# Autodesk Inventor assembly: x_carryage
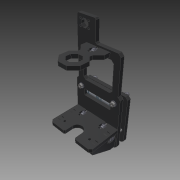
[picture p0: Inventor's stored thumbnail of the model, 180x180]
Saved by Autodesk Inventor 2014 (Build 180170000, 170)
## iProperties
Created: 2014-01-10
Part Number: x_carryage
Document SubType Name: Assembly
Designer: buben
Author: buben
## Documents named in this file (12)
- C:\Users\buben\Documents\GitHub\bacon\inventor files\assemblies\x_carryage.iam
- C:\Users\buben\Documents\GitHub\bacon\inventor files\printer parts\x_carriage_front.ipt
- C:\Users\buben\Documents\GitHub\bacon\inventor files\3rd party components\linear_bearing_8\Imported Components\LU8MM\LU8MM.iam
- C:\Users\buben\Documents\GitHub\bacon\inventor files\printer parts\x_carriage_back.ipt
- C:\Users\buben\Documents\GitHub\bacon\inventor files\printer parts\x_carriage_extruder_mount.ipt
- C:\Users\buben\Documents\GitHub\bacon\inventor files\printer parts\x_carryage_brace.ipt
- C:\Users\buben\Documents\GitHub\bacon\inventor files\printer parts\filament_guide.ipt
- C:\Users\buben\Documents\GitHub\bacon\inventor files\utils\washer_m4.ipt
- C:\Users\buben\Documents\Inventor\Content Center Files\R2014\en-US\ISO 4762(2)\ISO 4762 - M4 x 20ISO.ipt
- C:\Users\buben\Documents\Inventor\Content Center Files\R2014\en-US\ISO 4762(2)\ISO 4762 - M4 x 35ISO.ipt
- C:\Users\buben\Documents\Inventor\Content Center Files\R2014\en-US\ISO 4762(2)\ISO 4762 - M4 x 30ISO.ipt
- C:\Users\buben\Documents\Inventor\Content Center Files\R2014\en-US\ISO 7040\ISO 7040 - M4.ipt
## Components (41 placed, 11 different names)
1. x_carriage_front:1 — Flush:1, Mate:1, Mate:2, Mate:5, Mate:6, Mate:7, Mate:8, Mate:9, Mate:10, Mate:15, Mate:16, Mate:17, Mate:18, Mate:19, Mate:22, Mate:23, Mate:24, Mate:25, Mate:26, Mate:34, Mate:35, Mate:36, Mate:37, Mate:38, Mate:39, Mate:40, Mate:41
2. LU8MM:1 [sub-assembly] — Mate:8, Mate:9, Mate:10, Mate:13
3. LU8MM:2 [sub-assembly] — Mate:3, Mate:4, Mate:5, Mate:6
4. LU8MM:3 [sub-assembly] — Mate:3, Mate:4, Mate:7, Mate:11, Mate:12, Mate:14
5. x_carriage_back:1 — Mate:11, Mate:12, Mate:13, Mate:14, Mate:27, Mate:28, Mate:29, Mate:30, Mate:31, Mate:32, Mate:33, Mate:42, Mate:43, Mate:44, Mate:45
6. x_carriage_extruder_mount:1 — Mate:15, Mate:16, Mate:17, Mate:20, Mate:21, Mate:46, Mate:47
7. x_carryage_brace:1 — Mate:18, Mate:20, Mate:23, Mate:50
8. x_carryage_brace:2 — Mate:19, Mate:21, Mate:22, Mate:49
9. filament_guide:1 — Mate:24, Mate:25, Mate:26, Mate:48
10. CSN 02 1702 B B 4,3:1 — Mate:48, Mate:51, Mate:73
11. CSN 02 1702 B B 4,3:2 — Mate:34, Mate:35, Insert:1
12. CSN 02 1702 B B 4,3:3 — Mate:50, Mate:55, Mate:71
13. CSN 02 1702 B B 4,3:4 — Mate:38, Mate:39, Insert:4
14. CSN 02 1702 B B 4,3:5 — Mate:33, Mate:53, Mate:61
15. CSN 02 1702 B B 4,3:6 — Mate:32, Mate:54, Mate:63
16. CSN 02 1702 B B 4,3:7 — Mate:30, Mate:42, Insert:6
17. CSN 02 1702 B B 4,3:8 — Mate:36, Mate:37, Insert:3
18. CSN 02 1702 B B 4,3:9 — Mate:31, Mate:43, Insert:7
19. CSN 02 1702 B B 4,3:10 — Mate:49, Mate:58, Mate:65
20. CSN 02 1702 B B 4,3:11 — Mate:40, Mate:41, Insert:2
21. CSN 02 1702 B B 4,3:12 — Mate:47, Mate:56, Mate:69
22. CSN 02 1702 B B 4,3:13 — Mate:46, Mate:57, Mate:67
23. CSN 02 1702 B B 4,3:14 — Mate:29, Mate:44, Insert:8
24. CSN 02 1702 B B 4,3:15 — Mate:27, Mate:52, Mate:59
25. CSN 02 1702 B B 4,3:16 — Mate:28, Mate:45, Insert:5
26. ISO 4762 M4 x 30:2 — Insert:4, Mate:53, Mate:62
27. ISO 4762 M4 x 30:1 — Insert:3, Mate:54, Mate:64
28. ISO 4762 M4 x 20:3 — Insert:1, Mate:51, Mate:74
29. ISO 4762 M4 x 30:3 — Insert:2, Mate:52, Mate:60
30. ISO 4762 M4 x 35:1 — Insert:7, Mate:56, Mate:70
31. ISO 4762 M4 x 35:2 — Insert:8, Mate:55, Mate:72
32. ISO 4762 M4 x 35:3 — Insert:6, Mate:57, Mate:68
33. ISO 4762 M4 x 35:4 — Insert:5, Mate:58, Mate:66
34. DIN EN ISO 7040 M4:1 — Mate:63, Mate:64
35. DIN EN ISO 7040 M4:2 — Mate:69, Mate:70
36. DIN EN ISO 7040 M4:3 — Mate:67, Mate:68
37. DIN EN ISO 7040 M4:4 — Mate:59, Mate:60
38. DIN EN ISO 7040 M4:5 — Mate:65, Mate:66
39. DIN EN ISO 7040 M4:6 — Mate:61, Mate:62
40. DIN EN ISO 7040 M4:7 — Mate:73, Mate:74
41. DIN EN ISO 7040 M4:8 — Mate:71, Mate:72
## Relationships (83: Mate 74, Insert 8, Flush 1)
- Flush:1: x_carriage_front:1
- Mate:1: x_carriage_front:1
- Mate:2: x_carriage_front:1
- Mate:3: LU8MM:2 ↔ LU8MM:3
- Mate:4: LU8MM:2 ↔ LU8MM:3
- Mate:5 (7.5 mm): x_carriage_front:1 ↔ LU8MM:2
- Mate:6 (7.5 mm): x_carriage_front:1 ↔ LU8MM:2
- Mate:7 (0.5 mm): x_carriage_front:1 ↔ LU8MM:3
- Mate:8 (7.5 mm): x_carriage_front:1 ↔ LU8MM:1
- Mate:9 (7.5 mm): x_carriage_front:1 ↔ LU8MM:1
- Mate:10 (0.5 mm): x_carriage_front:1 ↔ LU8MM:1
- Mate:11 (7.5 mm): LU8MM:3 ↔ x_carriage_back:1
- Mate:12 (7.5 mm): LU8MM:3 ↔ x_carriage_back:1
- Mate:13 (7.5 mm): LU8MM:1 ↔ x_carriage_back:1
- Mate:14 (0.5 mm): LU8MM:3 ↔ x_carriage_back:1
- Mate:15: x_carriage_front:1 ↔ x_carriage_extruder_mount:1
- Mate:16: x_carriage_front:1 ↔ x_carriage_extruder_mount:1
- Mate:17: x_carriage_front:1 ↔ x_carriage_extruder_mount:1
- Mate:18: x_carriage_front:1 ↔ x_carryage_brace:1
- Mate:19: x_carriage_front:1 ↔ x_carryage_brace:2
- Mate:20: x_carriage_extruder_mount:1 ↔ x_carryage_brace:1
- Mate:21: x_carriage_extruder_mount:1 ↔ x_carryage_brace:2
- Mate:22: x_carriage_front:1 ↔ x_carryage_brace:2
- Mate:23: x_carriage_front:1 ↔ x_carryage_brace:1
- Mate:24: x_carriage_front:1 ↔ filament_guide:1
- Mate:25: x_carriage_front:1 ↔ filament_guide:1
- Mate:26: x_carriage_front:1 ↔ filament_guide:1
- Mate:27: x_carriage_back:1 ↔ CSN 02 1702 B B 4,3:15
- Mate:28: x_carriage_back:1 ↔ CSN 02 1702 B B 4,3:16
- Mate:29: x_carriage_back:1 ↔ CSN 02 1702 B B 4,3:14
- Mate:30: x_carriage_back:1 ↔ CSN 02 1702 B B 4,3:7
- Mate:31: x_carriage_back:1 ↔ CSN 02 1702 B B 4,3:9
- Mate:32: x_carriage_back:1 ↔ CSN 02 1702 B B 4,3:6
- Mate:33: x_carriage_back:1 ↔ CSN 02 1702 B B 4,3:5
- Mate:34: x_carriage_front:1 ↔ CSN 02 1702 B B 4,3:2
- Mate:35: x_carriage_front:1 ↔ CSN 02 1702 B B 4,3:2
- Mate:36: x_carriage_front:1 ↔ CSN 02 1702 B B 4,3:8
- Mate:37: x_carriage_front:1 ↔ CSN 02 1702 B B 4,3:8
- Mate:38: x_carriage_front:1 ↔ CSN 02 1702 B B 4,3:4
- Mate:39: x_carriage_front:1 ↔ CSN 02 1702 B B 4,3:4
- Mate:40: x_carriage_front:1 ↔ CSN 02 1702 B B 4,3:11
- Mate:41: x_carriage_front:1 ↔ CSN 02 1702 B B 4,3:11
- Mate:42: x_carriage_back:1 ↔ CSN 02 1702 B B 4,3:7
- Mate:43: x_carriage_back:1 ↔ CSN 02 1702 B B 4,3:9
- Mate:44: x_carriage_back:1 ↔ CSN 02 1702 B B 4,3:14
- Mate:45: x_carriage_back:1 ↔ CSN 02 1702 B B 4,3:16
- Mate:46: x_carriage_extruder_mount:1 ↔ CSN 02 1702 B B 4,3:13
- Mate:47: x_carriage_extruder_mount:1 ↔ CSN 02 1702 B B 4,3:12
- Mate:48: filament_guide:1 ↔ CSN 02 1702 B B 4,3:1
- Mate:49: x_carryage_brace:2 ↔ CSN 02 1702 B B 4,3:10
- Mate:50: x_carryage_brace:1 ↔ CSN 02 1702 B B 4,3:3
- Insert:1: CSN 02 1702 B B 4,3:2 ↔ ISO 4762 M4 x 20:3
- Insert:2: CSN 02 1702 B B 4,3:11 ↔ ISO 4762 M4 x 30:3
- Insert:3: CSN 02 1702 B B 4,3:8 ↔ ISO 4762 M4 x 30:1
- Insert:4: CSN 02 1702 B B 4,3:4 ↔ ISO 4762 M4 x 30:2
- Mate:51: CSN 02 1702 B B 4,3:1 ↔ ISO 4762 M4 x 20:3
- Mate:52: CSN 02 1702 B B 4,3:15 ↔ ISO 4762 M4 x 30:3
- Mate:53: CSN 02 1702 B B 4,3:5 ↔ ISO 4762 M4 x 30:2
- Mate:54: CSN 02 1702 B B 4,3:6 ↔ ISO 4762 M4 x 30:1
- Insert:5: CSN 02 1702 B B 4,3:16 ↔ ISO 4762 M4 x 35:4
- Insert:6: CSN 02 1702 B B 4,3:7 ↔ ISO 4762 M4 x 35:3
- Insert:7: CSN 02 1702 B B 4,3:9 ↔ ISO 4762 M4 x 35:1
- Insert:8: CSN 02 1702 B B 4,3:14 ↔ ISO 4762 M4 x 35:2
- Mate:55: CSN 02 1702 B B 4,3:3 ↔ ISO 4762 M4 x 35:2
- Mate:56: CSN 02 1702 B B 4,3:12 ↔ ISO 4762 M4 x 35:1
- Mate:57: CSN 02 1702 B B 4,3:13 ↔ ISO 4762 M4 x 35:3
- Mate:58: CSN 02 1702 B B 4,3:10 ↔ ISO 4762 M4 x 35:4
- Mate:59: CSN 02 1702 B B 4,3:15 ↔ DIN EN ISO 7040 M4:4
- Mate:60: ISO 4762 M4 x 30:3 ↔ DIN EN ISO 7040 M4:4
- Mate:61: CSN 02 1702 B B 4,3:5 ↔ DIN EN ISO 7040 M4:6
- Mate:62: ISO 4762 M4 x 30:2 ↔ DIN EN ISO 7040 M4:6
- Mate:63: CSN 02 1702 B B 4,3:6 ↔ DIN EN ISO 7040 M4:1
- Mate:64: ISO 4762 M4 x 30:1 ↔ DIN EN ISO 7040 M4:1
- Mate:65: CSN 02 1702 B B 4,3:10 ↔ DIN EN ISO 7040 M4:5
- Mate:66: ISO 4762 M4 x 35:4 ↔ DIN EN ISO 7040 M4:5
- Mate:67: CSN 02 1702 B B 4,3:13 ↔ DIN EN ISO 7040 M4:3
- Mate:68: ISO 4762 M4 x 35:3 ↔ DIN EN ISO 7040 M4:3
- Mate:69: CSN 02 1702 B B 4,3:12 ↔ DIN EN ISO 7040 M4:2
- Mate:70: ISO 4762 M4 x 35:1 ↔ DIN EN ISO 7040 M4:2
- Mate:71: CSN 02 1702 B B 4,3:3 ↔ DIN EN ISO 7040 M4:8
- Mate:72: ISO 4762 M4 x 35:2 ↔ DIN EN ISO 7040 M4:8
- Mate:73: CSN 02 1702 B B 4,3:1 ↔ DIN EN ISO 7040 M4:7
- Mate:74: ISO 4762 M4 x 20:3 ↔ DIN EN ISO 7040 M4:7
